# Autodesk Inventor assembly: Horizontal - Undercutter v0
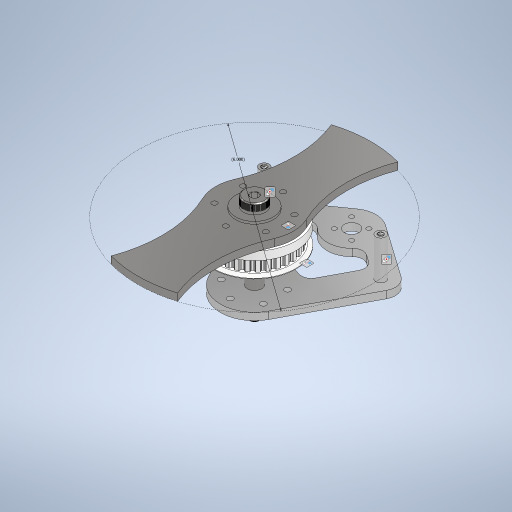
[picture p0: Inventor's stored thumbnail of the model, 512x512]
Saved by Autodesk Inventor 2023.4 (Build 274418000, 418)
## iProperties
Created: 2024-09-12
Part Number: Horizontal - Undercutter v0
Document SubType Name: Assembly
Designer: Nathan Cai
Author: Nathan Cai
## Documents named in this file (7)
- E:\Documents\Inventor\Law - V2.1\Horizontal - Undercutter V0\Horizontal - Undercutter v0.iam
- E:\Documents\Inventor\Law - V2.1\Horizontal - Undercutter V0\Upright - Bottom.ipt
- E:\Documents\Inventor\Law - V2.1\Horizontal - Undercutter V0\Blade (Bar 2).ipt
- E:\Documents\Inventor\Law - V2.1\Horizontal - Undercutter V0\XL Pulley Base.ipt
- E:\Documents\Inventor\Law - V2.1\Flange Bearing - 3-8x 7-8x 9-32.ipt
- E:\Documents\Inventor\Law - V2.1\Horizontal - Undercutter V0\91259A632_Alloy Steel Shoulder Screw.ipt
- E:\Documents\Inventor\Law - V2.1\Horizontal - Undercutter V0\Standoff 1in.ipt
## Components (8 placed, 6 different names)
1. Upright - Bottom:1 — Mate:1, Mate:2, Mate:3, Mate:4, Mate:12, Mate:15
2. Standoff 1in:1 — Mate:1, Mate:4
3. Standoff 1in:2 — Mate:2, Mate:3
4. Blade (Bar 2):1 — Mate:5, Mate:6, Mate:7, Mate:8, Mate:9
5. XL Pulley Base:1 — Mate:5, Mate:6, Mate:7, Mate:10, Mate:11
6. Flange Bearing - 3-8x 7-8x 9-32:1 — Mate:8, Mate:9, Mate:13, Mate:14
7. Flange Bearing - 3-8x 7-8x 9-32:2 — Mate:10, Mate:11, Mate:12, Mate:15
8. 91259A632_Alloy Steel Shoulder Screw:1 — Mate:13, Mate:14
## Relationships (15: Mate 15)
- Mate:1: Upright - Bottom:1 ↔ Standoff 1in:1
- Mate:2: Upright - Bottom:1 ↔ Standoff 1in:2
- Mate:3: Upright - Bottom:1 ↔ Standoff 1in:2
- Mate:4: Upright - Bottom:1 ↔ Standoff 1in:1
- Mate:5: Blade (Bar 2):1 ↔ XL Pulley Base:1
- Mate:6: Blade (Bar 2):1 ↔ XL Pulley Base:1
- Mate:7: Blade (Bar 2):1 ↔ XL Pulley Base:1
- Mate:8: Blade (Bar 2):1 ↔ Flange Bearing - 3-8x 7-8x 9-32:1
- Mate:9: Blade (Bar 2):1 ↔ Flange Bearing - 3-8x 7-8x 9-32:1
- Mate:10: XL Pulley Base:1 ↔ Flange Bearing - 3-8x 7-8x 9-32:2
- Mate:11: XL Pulley Base:1 ↔ Flange Bearing - 3-8x 7-8x 9-32:2
- Mate:12: Upright - Bottom:1 ↔ Flange Bearing - 3-8x 7-8x 9-32:2
- Mate:13: Flange Bearing - 3-8x 7-8x 9-32:1 ↔ 91259A632_Alloy Steel Shoulder Screw:1
- Mate:14: Flange Bearing - 3-8x 7-8x 9-32:1 ↔ 91259A632_Alloy Steel Shoulder Screw:1
- Mate:15 (20.6375 mm): Upright - Bottom:1 ↔ Flange Bearing - 3-8x 7-8x 9-32:2
